# Autodesk Inventor assembly: A_snap_001
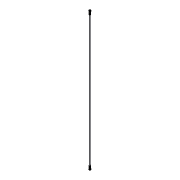
[picture p0: Inventor's stored thumbnail of the model, 180x180]
Saved by Autodesk Inventor 2016 (Build 200138000, 138)
## iProperties
Created: 2016-02-26
Part Number: A_snap_001
Document SubType Name: Assembly
Designer: Mateusz
Author: Mateusz
## Documents named in this file (3)
- D:\PROJECTS\2016_biped\hermes\mechanics_tmp\A_snap_001.iam
- D:\PROJECTS\2016_biped\hermes\mechanics_tmp\P_threaded_rod_M3_001.ipt
- D:\PROJECTS\2016_biped\hermes\mechanics_tmp\P_snap_001.ipt
## Components (3 placed, 2 different names)
1. P_threaded_rod_M3_001:1 — Mate:1, Mate:2, Mate:3, Mate:4
2. P_snap_001:1 — Mate:1, Mate:2
3. P_snap_001:2 — Mate:3, Mate:4
## Relationships (4: Mate 4)
- Mate:1: P_threaded_rod_M3_001:1 ↔ P_snap_001:1
- Mate:2 (-5 mm): P_threaded_rod_M3_001:1 ↔ P_snap_001:1
- Mate:3: P_threaded_rod_M3_001:1 ↔ P_snap_001:2
- Mate:4 (-8 mm): P_threaded_rod_M3_001:1 ↔ P_snap_001:2
